# Autodesk Inventor assembly: JOINT_20X20_detail
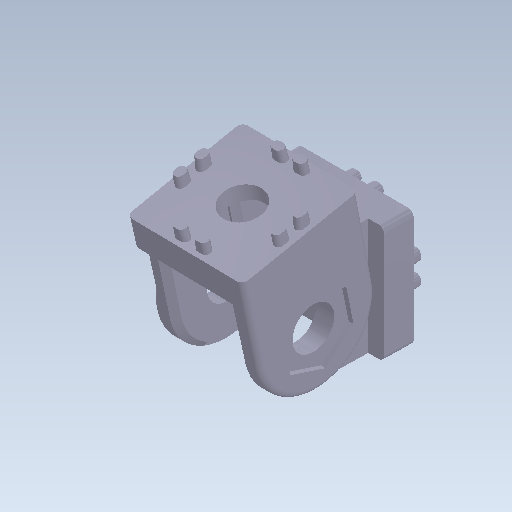
[picture p0: Inventor's stored thumbnail of the model, 512x512]
Saved by Autodesk Inventor 2021 (Build 250183000, 183)
## iProperties
Created: 2021-03-09
Part Number: JOINT_20X20_detail
Document SubType Name: Assembly
Designer: negt20
Sending System: Bosch Rexroth AG
Major Version: 4.0
Minor Version: 0.0
Format Version: 0.0
Product Id: Bosch Rexroth AG
Author: negt20
## Documents named in this file (13)
- C:\Users\negt20\OneDrive - University of Bath\Documents\Inventor\Pass_Fail_Rig\New Rig\JOINT_20X20_detail.iam
- C:\Users\negt20\OneDrive - University of Bath\Documents\Inventor\Pass_Fail_Rig\New Rig\Base Company Files\JOINT_20X20_detail.ipt
- C:\Users\negt20\OneDrive - University of Bath\Documents\Inventor\Pass_Fail_Rig\New Rig\Base Company Files\JOINT_20X20_detail_1.ipt
- C:\Users\negt20\OneDrive - University of Bath\Documents\Inventor\Pass_Fail_Rig\New Rig\Base Company Files\JOINT_20X20_detail_2.ipt
- C:\Users\negt20\OneDrive - University of Bath\Documents\Inventor\Pass_Fail_Rig\New Rig\Base Company Files\JOINT_20X20_detail_3.ipt
- C:\Users\negt20\OneDrive - University of Bath\Documents\Inventor\Pass_Fail_Rig\New Rig\Base Company Files\JOINT_20X20_detail_4.ipt
- C:\Users\negt20\OneDrive - University of Bath\Documents\Inventor\Pass_Fail_Rig\New Rig\Base Company Files\JOINT_20X20_detail_5.ipt
- C:\Users\negt20\OneDrive - University of Bath\Documents\Inventor\Pass_Fail_Rig\New Rig\Base Company Files\JOINT_20X20_detail_6.ipt
- C:\Users\negt20\OneDrive - University of Bath\Documents\Inventor\Pass_Fail_Rig\New Rig\Base Company Files\JOINT_20X20_detail_7.ipt
- C:\Users\negt20\OneDrive - University of Bath\Documents\Inventor\Pass_Fail_Rig\New Rig\Base Company Files\JOINT_20X20_detail_8.ipt
- C:\Users\negt20\OneDrive - University of Bath\Documents\Inventor\Pass_Fail_Rig\New Rig\Base Company Files\JOINT_20X20_detail_9.ipt
- C:\Users\negt20\OneDrive - University of Bath\Documents\Inventor\Pass_Fail_Rig\New Rig\Base Company Files\JOINT_20X20_detail_10.ipt
- C:\Users\negt20\OneDrive - University of Bath\Documents\Inventor\Pass_Fail_Rig\New Rig\Base Company Files\JOINT_20X20_detail_11.ipt
## Components (12 placed, 12 different names)
1. JOINT_20X20_detail_1:1
2. JOINT_20X20_detail_2:1 — Rotational:1
3. JOINT_20X20_detail_3:1
4. JOINT_20X20_detail_4:1
5. JOINT_20X20_detail_5:1
6. JOINT_20X20_detail_6:1
7. JOINT_20X20_detail_7:1
8. JOINT_20X20_detail_8:1
9. JOINT_20X20_detail_9:1
10. JOINT_20X20_detail_10:1
11. JOINT_20X20_detail_11:1
12. JOINT_20X20_detail_12:1 — Rotational:1
## Relationships (1: RevoluteJoint 1)
- Rotational:1 [RevoluteJoint]: JOINT_20X20_detail_2:1 ↔ JOINT_20X20_detail_12:1
